# Autodesk Inventor assembly: wszystkie scianki
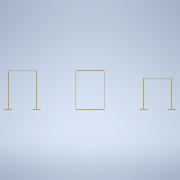
[picture p0: Inventor's stored thumbnail of the model, 180x180]
Saved by Autodesk Inventor 2021 (Build 250183000, 183)
## iProperties
Created: 2024-04-21
Part Number: wszystkie scianki
Document SubType Name: Assembly
Designer: Michal
Author: Michal
## Documents named in this file (4)
- C:\Users\Michal\Documents\GitHub\PNW_PhotoBoothFrame_3D\wszystkie scianki.iam
- C:\Users\Michal\Documents\GitHub\PNW_PhotoBoothFrame_3D\prostkatna waska wysoka kwadraty.iam
- C:\Users\Michal\Documents\GitHub\PNW_PhotoBoothFrame_3D\prostkatna waska wysoka lacznik.iam
- C:\Users\Michal\Documents\GitHub\PNW_PhotoBoothFrame_3D\prostkatna waska niska kwadraty.iam
## Components (3 placed, 3 different names)
1. prostkatna waska wysoka kwadraty:1 [sub-assembly] — Flush:1, Flush:2, Mate:1
2. prostkatna waska wysoka lacznik:1 [sub-assembly] — Flush:1, Flush:2, Mate:1, Flush:3, Flush:4, Mate:2
3. prostkatna waska niska kwadraty:1 [sub-assembly] — Flush:3, Flush:4, Mate:2
## Relationships (6: Flush 4, Mate 2)
- Flush:1: prostkatna waska wysoka kwadraty:1 ↔ prostkatna waska wysoka lacznik:1
- Flush:2: prostkatna waska wysoka kwadraty:1 ↔ prostkatna waska wysoka lacznik:1
- Mate:1 (2000 mm): prostkatna waska wysoka kwadraty:1 ↔ prostkatna waska wysoka lacznik:1
- Flush:3: prostkatna waska wysoka lacznik:1 ↔ prostkatna waska niska kwadraty:1
- Flush:4: prostkatna waska wysoka lacznik:1 ↔ prostkatna waska niska kwadraty:1
- Mate:2 (2000 mm): prostkatna waska wysoka lacznik:1 ↔ prostkatna waska niska kwadraty:1
